# Autodesk Inventor assembly: Assembly1
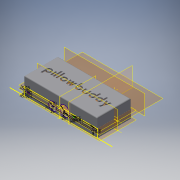
[picture p0: Inventor's stored thumbnail of the model, 180x180]
Saved by Autodesk Inventor 2019 (Build 230136000, 136)
## iProperties
Created: 2019-08-11
Part Number: Assembly1
Document SubType Name: Assembly
Designer: tmst0
Author: tmst0
## Documents named in this file (3)
- D:\RB\STL\Assembly1.iam
- D:\RB\STL\bottom.ipt
- D:\RB\STL\top_punched.ipt
## Components (2 placed, 2 different names)
1. bottom:1 — Mate:1
2. top_punched:1 — Mate:1
## Relationships (1: Mate 1)
- Mate:1: bottom:1 ↔ top_punched:1
